# Autodesk Inventor assembly: ButterBox
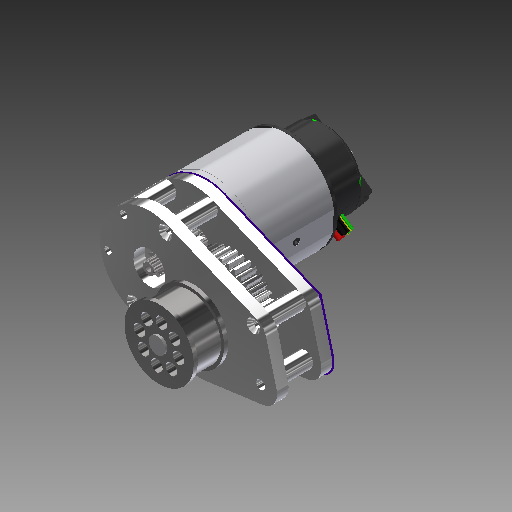
[picture p0: Inventor's stored thumbnail of the model, 512x512]
Saved by Autodesk Inventor 2019.4 (Build 234330000, 330)
## iProperties
Created: 2019-12-31
Part Number: ButterBox
Document SubType Name: Assembly
Designer: Mark
Mass: 967.976 g
Surface Area: 1147.69 cm^2
Volume: 273.494 cm^3
Density: 3.53929 g/cm^3
Author: Mark
## Documents named in this file (10)
- C:\Users\Mark\Desktop\7738 Helion Engineering\7738-CAD-prep\Butterfly Drive Mk3\ButterBox.iam
- C:\Users\Mark\Desktop\7738 Helion Engineering\7738-CAD-prep\Swerve Module\Falcon_500_Powered_by_Talon_FX_217-6515.iam
- C:\Users\Mark\Desktop\7738 Helion Engineering\7738-CAD-prep\Butterfly Drive Mk3\Inner Plate.ipt
- C:\Users\Mark\Desktop\7738 Helion Engineering\7738-CAD-prep\WCD\F63800.ipt
- C:\Users\Mark\Desktop\7738 Helion Engineering\7738-CAD-prep\WCD\10T_Steel_Spur_Gear_20_DP_12T_Center_Distance_Falcon_Motor_217-6917.ipt
- C:\Users\Mark\Desktop\7738 Helion Engineering\7738-CAD-prep\Offline CAD\MK3 Gearbox\40t_Aluminum_Spur_Gear_20_DP_1_2_Hex_Bore_217-2708.ipt
- C:\Users\Mark\Desktop\7738 Helion Engineering\7738-CAD-prep\Butterfly Drive Mk3\Gearbox Spacer.ipt
- C:\Users\Mark\Desktop\7738 Helion Engineering\7738-CAD-prep\Butterfly Drive Mk3\ButterBox\Design Accelerator\Shaft1.iam
- C:\Users\Mark\Desktop\7738 Helion Engineering\7738-CAD-prep\Butterfly Drive Mk3\24 Teeth HTD5M Pulley Steel.ipt
- C:\Users\Mark\Desktop\7738 Helion Engineering\7738-CAD-prep\Butterfly Drive Mk3\Outer Plate.ipt
## Components (16 placed, 9 different names)
1. Falcon_500_Powered_by_Talon_FX_217-6515:1 [sub-assembly] — Mate:1, Mate:2, Mate:5
2. Inner Plate:1 — Mate:1, Mate:2, Mate:3, Mate:4, Mate:6, Mate:11, Mate:15, Mate:16, Mate:19, Mate:20, Mate:21, Mate:22, Flush:3, Mate:26, Mate:27, Mate:28, Mate:29, Mate:30, Mate:31, Mate:32, Flush:4, Flush:5
3. F63800:1 — Mate:3, Mate:4, Mate:7, Mate:8, Mate:9, Mate:23
4. 10T_Steel_Spur_Gear_20_DP_12T_Center_Distance_Falcon_Motor_217-6917:1 — Mate:5, Mate:6
5. 40t_Aluminum_Spur_Gear_20_DP_1_2_Hex_Bore_217-2708:1 — Mate:7, Mate:8
6. F63800:2 — Mate:9, Mate:11
7. Gearbox Spacer:1
8. Gearbox Spacer:2 — Mate:15, Mate:16
9. Gearbox Spacer:3 — Mate:28, Mate:29
10. Gearbox Spacer:4 — Mate:19, Mate:20
11. Gearbox Spacer:5 — Mate:21, Mate:22
12. Shaft:1 [sub-assembly] — Mate:23, Flush:3, Mate:24
13. 24 Teeth HTD5M Pulley Steel:1 — Mate:24
14. Gearbox Spacer:6 — Mate:26, Mate:27
15. Gearbox Spacer:7 — Mate:30, Mate:31
16. Outer Plate:1 — Mate:32, Flush:4, Flush:5
## Relationships (28: Mate 25, Flush 3)
- Mate:1: Falcon_500_Powered_by_Talon_FX_217-6515:1 ↔ Inner Plate:1
- Mate:2: Falcon_500_Powered_by_Talon_FX_217-6515:1 ↔ Inner Plate:1
- Mate:3: Inner Plate:1 ↔ F63800:1
- Mate:4: Inner Plate:1 ↔ F63800:1
- Mate:5: Falcon_500_Powered_by_Talon_FX_217-6515:1 ↔ 10T_Steel_Spur_Gear_20_DP_12T_Center_Distance_Falcon_Motor_217-6917:1
- Mate:6: Inner Plate:1 ↔ 10T_Steel_Spur_Gear_20_DP_12T_Center_Distance_Falcon_Motor_217-6917:1
- Mate:7: F63800:1 ↔ 40t_Aluminum_Spur_Gear_20_DP_1_2_Hex_Bore_217-2708:1
- Mate:8 (2.1755 mm): F63800:1 ↔ 40t_Aluminum_Spur_Gear_20_DP_1_2_Hex_Bore_217-2708:1
- Mate:9: F63800:1 ↔ F63800:2
- Mate:11 (18.5 mm): Inner Plate:1 ↔ F63800:2
- Mate:15: Inner Plate:1 ↔ Gearbox Spacer:2
- Mate:16: Inner Plate:1 ↔ Gearbox Spacer:2
- Mate:19: Inner Plate:1 ↔ Gearbox Spacer:4
- Mate:20: Inner Plate:1 ↔ Gearbox Spacer:4
- Mate:21: Inner Plate:1 ↔ Gearbox Spacer:5
- Mate:22: Inner Plate:1 ↔ Gearbox Spacer:5
- Mate:23: F63800:1 ↔ Shaft:1
- Flush:3 (0.5 mm): Inner Plate:1 ↔ Shaft:1
- Mate:24: Shaft:1 ↔ 24 Teeth HTD5M Pulley Steel:1
- Mate:26: Inner Plate:1 ↔ Gearbox Spacer:6
- Mate:27: Inner Plate:1 ↔ Gearbox Spacer:6
- Mate:28: Inner Plate:1 ↔ Gearbox Spacer:3
- Mate:29: Inner Plate:1 ↔ Gearbox Spacer:3
- Mate:30: Inner Plate:1 ↔ Gearbox Spacer:7
- Mate:31: Inner Plate:1 ↔ Gearbox Spacer:7
- Mate:32 (20 mm): Inner Plate:1 ↔ Outer Plate:1
- Flush:4: Inner Plate:1 ↔ Outer Plate:1
- Flush:5: Inner Plate:1 ↔ Outer Plate:1
